# Autodesk Inventor assembly: Cámara de profundidad
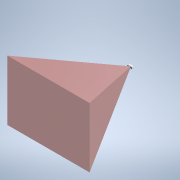
[picture p0: Inventor's stored thumbnail of the model, 180x180]
Saved by Autodesk Inventor 2022.1 (Build 261234000, 234)
## iProperties
Created: 2021-10-01
Part Number: Cámara de profundidad
Document SubType Name: Assembly
Designer: seb_0
Author: seb_0
## Documents named in this file (4)
- C:\Users\seb_0\Desktop\PDM\ProyectoRobotPallet\Cámara de profundidad\Cámara de profundidad.iam
- C:\Users\seb_0\Desktop\PDM\ProyectoRobotPallet\Cámara de profundidad\Intel_RealSense_Depth_Camera_D435.ipt
- C:\Users\seb_0\Desktop\PDM\ProyectoRobotPallet\Cámara de profundidad\Soporte_Cámara.ipt
- C:\Users\seb_0\Desktop\PDM\ProyectoRobotPallet\Cámara de profundidad\Visión_Cámara.ipt
## Components (3 placed, 3 different names)
1. Intel_RealSense_Depth_Camera_D435:1 — Coincidencia:3, Coincidencia:4, Coincidencia:5, Coincidencia:6
2. Soporte_Cámara:1 — Coincidencia:1, Coincidencia:2, Coincidencia:3, Coincidencia:4, Coincidencia:5, Coincidencia:7, Coincidencia:8
3. Visión_Cámara:1 — Coincidencia:6, Coincidencia:7, Coincidencia:8
## Relationships (8: Mate 8)
- Coincidencia:1 [Mate]: Soporte_Cámara:1
- Coincidencia:2 [Mate]: Soporte_Cámara:1
- Coincidencia:3 [Mate]: Intel_RealSense_Depth_Camera_D435:1 ↔ Soporte_Cámara:1
- Coincidencia:4 [Mate]: Intel_RealSense_Depth_Camera_D435:1 ↔ Soporte_Cámara:1
- Coincidencia:5 [Mate]: Intel_RealSense_Depth_Camera_D435:1 ↔ Soporte_Cámara:1
- Coincidencia:6 [Mate]: Intel_RealSense_Depth_Camera_D435:1 ↔ Visión_Cámara:1
- Coincidencia:7 [Mate] (-10.125 mm): Soporte_Cámara:1 ↔ Visión_Cámara:1
- Coincidencia:8 [Mate] (-20.26 mm): Soporte_Cámara:1 ↔ Visión_Cámara:1
